# Autodesk Inventor assembly: enix_assembly_v2
(part 2 of 2)
- Mate:543: baseplate:1 ↔ AS 1427 H - Metric M2 x 8:49
- Mate:544: baseplate:1 ↔ AS 1427 H - Metric M2 x 8:49
- Mate:545: baseplate:1 ↔ AS 1427 H - Metric M2 x 8:50
- Mate:546: battery_distancer:2 ↔ AS 1112 (2) - Metric M2  Type 5:54
- Mate:547: AS 1427 H - Metric M2 x 8:50 ↔ AS 1112 (2) - Metric M2  Type 5:54
- Mate:548: battery_distancer:1 ↔ AS 1112 (2) - Metric M2  Type 5:53
- Mate:549: AS 1427 H - Metric M2 x 8:49 ↔ AS 1112 (2) - Metric M2  Type 5:53
- Mate:550: battery_distancer:1 ↔ AS 1112 (2) - Metric M2  Type 5:52
- Mate:551: AS 1427 H - Metric M2 x 8:48 ↔ AS 1112 (2) - Metric M2  Type 5:52
- Mate:552: battery_distancer:2 ↔ AS 1112 (2) - Metric M2  Type 5:51
- Mate:553: AS 1427 H - Metric M2 x 8:47 ↔ AS 1112 (2) - Metric M2  Type 5:51
- Mate:554: battery_distancer:2 ↔ battery_vant_4500_4s:1
- Mate:555 (1 mm): battery_distancer:2 ↔ battery_vant_4500_4s:1
- Mate:556: transformer:1 ↔ AS 1427 H - Metric M2 x 8:51
- Mate:557: transformer:1 ↔ AS 1427 H - Metric M2 x 8:52
- Mate:558: transformer:1 ↔ AS 1427 H - Metric M2 x 8:52
- Mate:559: transformer:1 ↔ AS 1427 H - Metric M2 x 8:51
- Mate:560: transformer:2 ↔ AS 1427 H - Metric M2 x 8:54
- Mate:561: transformer:2 ↔ AS 1427 H - Metric M2 x 8:53
- Mate:562: transformer:2 ↔ AS 1427 H - Metric M2 x 8:53
- Mate:563: transformer:2 ↔ AS 1427 H - Metric M2 x 8:54
- Mate:564: arm_back_rect:2 ↔ motor_mount_lock:4
- Mate:565: arm_front_rect:2 ↔ motor_mount_lock:1
- Mate:566: arm_front_rect:1 ↔ motor_mount_lock:2
- Mate:567: arm_back_rect:1 ↔ motor_mount_lock:3
- Mate:568: arm_back_rect:2 ↔ arm_socket_l:1
- Mate:569: arm_back_rect:2 ↔ arm_socket_l:1
- Mate:570 (0.05 mm): arm_back_rect:2 ↔ arm_socket_l:1
- Mate:571: arm_front_rect:2 ↔ arm_socket_l:2
- Mate:572: arm_front_rect:2 ↔ arm_socket_l:2
- Mate:573 (0.05 mm): arm_front_rect:2 ↔ arm_socket_l:2
- Mate:574: baseplate:1 ↔ arm_socket_l:1
- Mate:575: baseplate:1 ↔ arm_socket_l:1
- Angle:9 (0 deg): baseplate:1 ↔ arm_back_rect:2
- Mate:576: baseplate:1 ↔ arm_socket_l:2
- Mate:577: baseplate:1 ↔ arm_socket_l:2
- Angle:10 (0 deg): baseplate:1 ↔ arm_front_rect:2
- Mate:578: arm_back_rect:1 ↔ arm_socket_r:1
- Mate:579 (0.05 mm): arm_back_rect:1 ↔ arm_socket_r:1
- Mate:580: arm_back_rect:1 ↔ arm_socket_r:1
- Mate:581: arm_front_rect:1 ↔ arm_socket_r:2
- Mate:582 (0.05 mm): arm_front_rect:1 ↔ arm_socket_r:2
- Mate:583: arm_front_rect:1 ↔ arm_socket_r:2
- Mate:584: baseplate:1 ↔ arm_socket_r:2
- Mate:585: baseplate:1 ↔ arm_socket_r:2
- Angle:11 (0 deg): baseplate:1 ↔ arm_front_rect:1
- Mate:586: baseplate:1 ↔ arm_socket_r:1
- Mate:587: baseplate:1 ↔ arm_socket_r:1
- Angle:12 (0 deg): baseplate:1 ↔ arm_back_rect:1
- Mate:588: motor_mount:2 ↔ AS 1112 (2) - Metric M2  Type 5:55
- Mate:589: motor_mount:2 ↔ AS 1112 (2) - Metric M2  Type 5:55
- Mate:590: motor_mount:2 ↔ AS 1112 (2) - Metric M2  Type 5:56
- Mate:591: motor_mount:2 ↔ AS 1112 (2) - Metric M2  Type 5:56
- Mate:592: motor_mount:1 ↔ AS 1112 (2) - Metric M2  Type 5:61
- Mate:593: motor_mount:1 ↔ AS 1112 (2) - Metric M2  Type 5:61
- Mate:594: motor_mount:1 ↔ AS 1112 (2) - Metric M2  Type 5:62
- Mate:595: motor_mount:1 ↔ AS 1112 (2) - Metric M2  Type 5:62
- Mate:596: motor_mount:4 ↔ AS 1112 (2) - Metric M2  Type 5:60
- Mate:597: motor_mount:4 ↔ AS 1112 (2) - Metric M2  Type 5:60
- Mate:598: motor_mount:4 ↔ AS 1112 (2) - Metric M2  Type 5:59
- Mate:599: motor_mount:4 ↔ AS 1112 (2) - Metric M2  Type 5:59
- Mate:600: motor_mount:3 ↔ AS 1112 (2) - Metric M2  Type 5:57
- Mate:601: motor_mount:3 ↔ AS 1112 (2) - Metric M2  Type 5:57
- Mate:602: motor_mount:3 ↔ AS 1112 (2) - Metric M2  Type 5:58
- Mate:603: motor_mount:3 ↔ AS 1112 (2) - Metric M2  Type 5:58
- Mate:604: motor_mount_lock:3 ↔ AS 1427 H - Metric M2 x 12:1
- Mate:605: motor_mount_lock:3 ↔ AS 1427 H - Metric M2 x 12:1
- Mate:606: motor_mount_lock:3 ↔ AS 1427 H - Metric M2 x 12:2
- Mate:607: motor_mount_lock:3 ↔ AS 1427 H - Metric M2 x 12:2
- Mate:608: motor_mount_lock:4 ↔ AS 1427 H - Metric M2 x 12:5
- Mate:609: motor_mount_lock:4 ↔ AS 1427 H - Metric M2 x 12:5
- Mate:610: motor_mount_lock:4 ↔ AS 1427 H - Metric M2 x 12:6
- Mate:611: motor_mount_lock:4 ↔ AS 1427 H - Metric M2 x 12:6
- Mate:612: motor_mount_lock:1 ↔ AS 1427 H - Metric M2 x 12:8
- Mate:613: motor_mount_lock:1 ↔ AS 1427 H - Metric M2 x 12:8
- Mate:614: motor_mount_lock:1 ↔ AS 1427 H - Metric M2 x 12:7
- Mate:615: motor_mount_lock:1 ↔ AS 1427 H - Metric M2 x 12:7
- Mate:616: motor_mount_lock:2 ↔ AS 1427 H - Metric M2 x 12:3
- Mate:617: motor_mount_lock:2 ↔ AS 1427 H - Metric M2 x 12:3
- Mate:618: motor_mount_lock:2 ↔ AS 1427 H - Metric M2 x 12:4
- Mate:619: motor_mount_lock:2 ↔ AS 1427 H - Metric M2 x 12:4
- Mate:620: motor_mount_lock:2 ↔ AS 1427 H - Metric M3 x 10:1
- Mate:621: motor_mount_lock:2 ↔ AS 1427 H - Metric M3 x 10:1
- Mate:622: arm_front_rect:1 ↔ ANSI B18.2.4.2M M3x0,5:1
- Mate:623: AS 1427 H - Metric M3 x 10:1 ↔ ANSI B18.2.4.2M M3x0,5:1
- Mate:624: motor_mount_lock:3 ↔ AS 1427 H - Metric M3 x 10:2
- Mate:625: motor_mount_lock:3 ↔ AS 1427 H - Metric M3 x 10:2
- Mate:626: motor_mount_lock:4 ↔ AS 1427 H - Metric M3 x 10:3
- Mate:627: motor_mount_lock:4 ↔ AS 1427 H - Metric M3 x 10:3
- Mate:628: motor_mount_lock:1 ↔ AS 1427 H - Metric M3 x 10:4
- Mate:629: motor_mount_lock:1 ↔ AS 1427 H - Metric M3 x 10:4
- Mate:630: arm_back_rect:1 ↔ ANSI B18.2.4.2M M3x0,5:2
- Mate:631: AS 1427 H - Metric M3 x 10:2 ↔ ANSI B18.2.4.2M M3x0,5:2
- Mate:632: arm_back_rect:2 ↔ ANSI B18.2.4.2M M3x0,5:3
- Mate:633: AS 1427 H - Metric M3 x 10:3 ↔ ANSI B18.2.4.2M M3x0,5:3
- Mate:634: arm_front_rect:2 ↔ ANSI B18.2.4.2M M3x0,5:4
- Mate:635: AS 1427 H - Metric M3 x 10:4 ↔ ANSI B18.2.4.2M M3x0,5:4
- Mate:636: motor_mount:3 ↔ Emax Rs2205 v1:4
- Mate:637: motor_mount:3 ↔ Emax Rs2205 v1:4
- Mate:638: motor_mount:3 ↔ Emax Rs2205 v1:4
- Mate:639: motor_mount:3 ↔ AS 1427 H - Metric M3 x 5:21
- Mate:640: motor_mount:3 ↔ AS 1427 H - Metric M3 x 5:21
- Mate:641: motor_mount:3 ↔ AS 1427 H - Metric M3 x 5:24
- Mate:642: motor_mount:3 ↔ AS 1427 H - Metric M3 x 5:24
- Mate:643: motor_mount:3 ↔ AS 1427 H - Metric M3 x 5:23
- Mate:644: motor_mount:3 ↔ AS 1427 H - Metric M3 x 5:23
- Mate:645: motor_mount:3 ↔ AS 1427 H - Metric M3 x 5:22
- Mate:646: motor_mount:3 ↔ AS 1427 H - Metric M3 x 5:22
- Mate:647: motor_mount:4 ↔ AS 1427 H - Metric M3 x 5:33
- Mate:648: motor_mount:4 ↔ AS 1427 H - Metric M3 x 5:33
- Mate:649: motor_mount:4 ↔ AS 1427 H - Metric M3 x 5:34
- Mate:650: motor_mount:4 ↔ AS 1427 H - Metric M3 x 5:34
- Mate:651: motor_mount:4 ↔ AS 1427 H - Metric M3 x 5:35
- Mate:652: motor_mount:4 ↔ AS 1427 H - Metric M3 x 5:35
- Mate:653: motor_mount:4 ↔ AS 1427 H - Metric M3 x 5:36
- Mate:654: motor_mount:4 ↔ AS 1427 H - Metric M3 x 5:36
- Mate:655: motor_mount:4 ↔ Emax Rs2205 v1:3
- Mate:656: Emax Rs2205 v1:3 ↔ AS 1427 H - Metric M3 x 5:33
- Mate:657: Emax Rs2205 v1:3 ↔ AS 1427 H - Metric M3 x 5:34
- Mate:658: motor_mount:1 ↔ AS 1427 H - Metric M3 x 5:27
- Mate:659: motor_mount:1 ↔ AS 1427 H - Metric M3 x 5:26
- Mate:660: motor_mount:1 ↔ AS 1427 H - Metric M3 x 5:25
- Mate:661: motor_mount:1 ↔ AS 1427 H - Metric M3 x 5:28
- Mate:662: motor_mount:1 ↔ AS 1427 H - Metric M3 x 5:27
- Mate:663: motor_mount:1 ↔ AS 1427 H - Metric M3 x 5:26
- Mate:664: motor_mount:1 ↔ AS 1427 H - Metric M3 x 5:25
- Mate:665: motor_mount:1 ↔ AS 1427 H - Metric M3 x 5:28
- Mate:666: motor_mount:1 ↔ Emax Rs2205 v1:2
- Mate:667: Emax Rs2205 v1:2 ↔ AS 1427 H - Metric M3 x 5:26
- Mate:668: Emax Rs2205 v1:2 ↔ AS 1427 H - Metric M3 x 5:27
- Mate:669: motor_mount:2 ↔ AS 1427 H - Metric M3 x 5:31
- Mate:670: motor_mount:2 ↔ AS 1427 H - Metric M3 x 5:32
- Mate:671: motor_mount:2 ↔ AS 1427 H - Metric M3 x 5:29
- Mate:672: motor_mount:2 ↔ AS 1427 H - Metric M3 x 5:30
- Mate:673: motor_mount:2 ↔ AS 1427 H - Metric M3 x 5:30
- Mate:674: motor_mount:2 ↔ AS 1427 H - Metric M3 x 5:31
- Mate:675: motor_mount:2 ↔ AS 1427 H - Metric M3 x 5:29
- Mate:676: motor_mount:2 ↔ AS 1427 H - Metric M3 x 5:32
- Mate:677: motor_mount:2 ↔ Emax Rs2205 v1:1
- Mate:678: Emax Rs2205 v1:1 ↔ AS 1427 H - Metric M3 x 5:32
- Mate:679: Emax Rs2205 v1:1 ↔ AS 1427 H - Metric M3 x 5:29
- Mate:680: top_plate:1 ↔ AS 1427 H - Metric M2 x 8:55
- Mate:681: top_plate:1 ↔ AS 1427 H - Metric M2 x 8:57
- Mate:682: top_plate:1 ↔ AS 1427 H - Metric M2 x 8:56
- Mate:683: top_plate:1 ↔ AS 1427 H - Metric M2 x 8:59
- Mate:684: arm_socket_l:1 ↔ AS 1427 H - Metric M2 x 8:58
- Mate:685: arm_socket_l:1 ↔ AS 1427 H - Metric M2 x 8:60
- Mate:686: arm_socket_l:2 ↔ AS 1427 H - Metric M2 x 8:62
- Mate:687: arm_socket_l:2 ↔ AS 1427 H - Metric M2 x 8:61
- Mate:688: arm_socket_l:2 ↔ AS 1427 H - Metric M2 x 8:61
- Mate:689: arm_socket_l:2 ↔ AS 1427 H - Metric M2 x 8:62
- Mate:690: top_plate:1 ↔ AS 1427 H - Metric M2 x 8:55
- Mate:691: top_plate:1 ↔ AS 1427 H - Metric M2 x 8:57
- Mate:692: top_plate:1 ↔ AS 1427 H - Metric M2 x 8:69
- Mate:693: top_plate:1 ↔ AS 1427 H - Metric M2 x 8:70
- Mate:694: arm_socket_r:2 ↔ AS 1427 H - Metric M2 x 8:68
- Mate:695: arm_socket_r:2 ↔ AS 1427 H - Metric M2 x 8:67
- Mate:696: top_plate:1 ↔ AS 1427 H - Metric M2 x 8:66
- Mate:697: top_plate:1 ↔ AS 1427 H - Metric M2 x 8:65
- Mate:698: arm_socket_r:1 ↔ AS 1427 H - Metric M2 x 8:64
- Mate:699: arm_socket_r:1 ↔ AS 1427 H - Metric M2 x 8:63
- Mate:700: arm_socket_r:1 ↔ AS 1427 H - Metric M2 x 8:64
- Mate:701: top_plate:1 ↔ AS 1427 H - Metric M2 x 8:66
- Mate:702: top_plate:1 ↔ AS 1427 H - Metric M2 x 8:65
- Mate:703: arm_socket_r:1 ↔ AS 1427 H - Metric M2 x 8:63
- Mate:704: top_plate:1 ↔ AS 1427 H - Metric M2 x 8:59
- Mate:705: top_plate:1 ↔ AS 1427 H - Metric M2 x 8:56
- Mate:706: arm_socket_l:1 ↔ AS 1427 H - Metric M2 x 8:58
- Mate:707: arm_socket_l:1 ↔ AS 1427 H - Metric M2 x 8:60
- Mate:708: top_plate:1 ↔ AS 1427 H - Metric M2 x 8:70
- Mate:709: top_plate:1 ↔ AS 1427 H - Metric M2 x 8:69
- Mate:710: arm_socket_r:2 ↔ AS 1427 H - Metric M2 x 8:68
- Mate:711: arm_socket_r:2 ↔ AS 1427 H - Metric M2 x 8:67
- Mate:712: baseplate:1 ↔ AS 1112 (2) - Metric M2  Type 5:66
- Mate:713: baseplate:1 ↔ AS 1112 (2) - Metric M2  Type 5:65
- Mate:714: AS 1427 H - Metric M2 x 8:63 ↔ AS 1112 (2) - Metric M2  Type 5:65
- Mate:715: AS 1427 H - Metric M2 x 8:64 ↔ AS 1112 (2) - Metric M2  Type 5:66
- Mate:716: arm_socket_r:1 ↔ AS 1112 (2) - Metric M2  Type 5:64
- Mate:717: AS 1427 H - Metric M2 x 8:66 ↔ AS 1112 (2) - Metric M2  Type 5:64
- Mate:718: arm_socket_r:1 ↔ AS 1112 (2) - Metric M2  Type 5:63
- Mate:719: AS 1427 H - Metric M2 x 8:65 ↔ AS 1112 (2) - Metric M2  Type 5:63
- Mate:720: arm_socket_r:2 ↔ AS 1112 (2) - Metric M2  Type 5:67
- Mate:721: AS 1427 H - Metric M2 x 8:69 ↔ AS 1112 (2) - Metric M2  Type 5:67
- Mate:722: arm_socket_r:2 ↔ AS 1112 (2) - Metric M2  Type 5:70
- Mate:723: AS 1427 H - Metric M2 x 8:70 ↔ AS 1112 (2) - Metric M2  Type 5:70
- Mate:724: baseplate:1 ↔ AS 1112 (2) - Metric M2  Type 5:69
- Mate:725: baseplate:1 ↔ AS 1112 (2) - Metric M2  Type 5:68
- Mate:726: AS 1427 H - Metric M2 x 8:67 ↔ AS 1112 (2) - Metric M2  Type 5:68
- Mate:727: AS 1427 H - Metric M2 x 8:68 ↔ AS 1112 (2) - Metric M2  Type 5:69
- Mate:728: arm_socket_l:1 ↔ AS 1112 (2) - Metric M2  Type 5:77
- Mate:729: AS 1427 H - Metric M2 x 8:56 ↔ AS 1112 (2) - Metric M2  Type 5:77
- Mate:730: arm_socket_l:1 ↔ AS 1112 (2) - Metric M2  Type 5:75
- Mate:731: AS 1427 H - Metric M2 x 8:59 ↔ AS 1112 (2) - Metric M2  Type 5:75
- Mate:732: baseplate:1 ↔ AS 1112 (2) - Metric M2  Type 5:78
- Mate:733: baseplate:1 ↔ AS 1112 (2) - Metric M2  Type 5:76
- Mate:734: AS 1427 H - Metric M2 x 8:60 ↔ AS 1112 (2) - Metric M2  Type 5:76
- Mate:735: AS 1427 H - Metric M2 x 8:58 ↔ AS 1112 (2) - Metric M2  Type 5:78
- Mate:736: arm_socket_l:2 ↔ AS 1112 (2) - Metric M2  Type 5:71
- Mate:737: AS 1427 H - Metric M2 x 8:55 ↔ AS 1112 (2) - Metric M2  Type 5:71
- Mate:738: baseplate:1 ↔ AS 1112 (2) - Metric M2  Type 5:72
- Mate:739: AS 1427 H - Metric M2 x 8:62 ↔ AS 1112 (2) - Metric M2  Type 5:72
- Mate:740: baseplate:1 ↔ AS 1112 (2) - Metric M2  Type 5:74
- Mate:741: AS 1427 H - Metric M2 x 8:61 ↔ AS 1112 (2) - Metric M2  Type 5:74
- Mate:742: arm_socket_l:2 ↔ AS 1112 (2) - Metric M2  Type 5:73
- Mate:743: AS 1427 H - Metric M2 x 8:57 ↔ AS 1112 (2) - Metric M2  Type 5:73
- Mate:744: top_plate:1 ↔ AS 1427 H - Metric M3 x 30:1
- Mate:745: top_plate:1 ↔ AS 1427 H - Metric M3 x 30:1
- Mate:746: top_plate:1 ↔ AS 1427 H - Metric M3 x 30:2
- Mate:747: top_plate:1 ↔ AS 1427 H - Metric M3 x 30:4
- Mate:748: top_plate:1 ↔ AS 1427 H - Metric M3 x 30:3
- Mate:749: top_plate:1 ↔ AS 1427 H - Metric M3 x 30:3
- Mate:750: top_plate:1 ↔ AS 1427 H - Metric M3 x 30:4
- Mate:751: top_plate:1 ↔ AS 1427 H - Metric M3 x 30:2
- Mate:752: baseplate:1 ↔ ANSI B18.2.4.2M M3x0,5:8
- Mate:753: baseplate:1 ↔ ANSI B18.2.4.2M M3x0,5:6
- Mate:754: AS 1427 H - Metric M3 x 30:2 ↔ ANSI B18.2.4.2M M3x0,5:6
- Mate:755: AS 1427 H - Metric M3 x 30:1 ↔ ANSI B18.2.4.2M M3x0,5:8
- Mate:756: baseplate:1 ↔ ANSI B18.2.4.2M M3x0,5:5
- Mate:757: baseplate:1 ↔ ANSI B18.2.4.2M M3x0,5:5
- Mate:758: baseplate:1 ↔ ANSI B18.2.4.2M M3x0,5:7
- Mate:759: AS 1427 H - Metric M3 x 30:4 ↔ ANSI B18.2.4.2M M3x0,5:7
- Mate:760: top_plate:1 ↔ klatka_na_rpi:1
- Mate:761: top_plate:1 ↔ klatka_na_rpi:1
- Mate:762: top_plate:1 ↔ klatka_na_rpi:1
- Mate:763: top_plate:1 ↔ klatka_na_rpi:1
- Mate:764: klatka_na_rpi:1 ↔ AS 1427 H - Metric M2 x 8:73
- Mate:765: klatka_na_rpi:1 ↔ AS 1427 H - Metric M2 x 8:72
- Mate:766: klatka_na_rpi:1 ↔ AS 1427 H - Metric M2 x 8:71
- Mate:767: klatka_na_rpi:1 ↔ AS 1427 H - Metric M2 x 8:71
- Mate:768: klatka_na_rpi:1 ↔ AS 1427 H - Metric M2 x 8:72
- Mate:769: klatka_na_rpi:1 ↔ AS 1427 H - Metric M2 x 8:73
- Mate:770: klatka_na_rpi:1 ↔ AS 1427 H - Metric M2 x 8:76
- Mate:771: klatka_na_rpi:1 ↔ AS 1427 H - Metric M2 x 8:75
- Mate:772: klatka_na_rpi:1 ↔ AS 1427 H - Metric M2 x 8:74
- Mate:773: klatka_na_rpi:1 ↔ AS 1427 H - Metric M2 x 8:74
- Mate:774: klatka_na_rpi:1 ↔ AS 1427 H - Metric M2 x 8:75
- Mate:775: klatka_na_rpi:1 ↔ AS 1427 H - Metric M2 x 8:76
- Mate:776: top_plate:1 ↔ AS 1112 (2) - Metric M2  Type 5:80
- Mate:777: AS 1427 H - Metric M2 x 8:72 ↔ AS 1112 (2) - Metric M2  Type 5:80
- Mate:778: top_plate:1 ↔ AS 1112 (2) - Metric M2  Type 5:81
- Mate:779: AS 1427 H - Metric M2 x 8:71 ↔ AS 1112 (2) - Metric M2  Type 5:81
- Mate:780: top_plate:1 ↔ AS 1112 (2) - Metric M2  Type 5:79
- Mate:781: AS 1427 H - Metric M2 x 8:73 ↔ AS 1112 (2) - Metric M2  Type 5:79
- Mate:782: top_plate:1 ↔ AS 1112 (2) - Metric M2  Type 5:84
- Mate:783: AS 1427 H - Metric M2 x 8:76 ↔ AS 1112 (2) - Metric M2  Type 5:84
- Mate:784: top_plate:1 ↔ AS 1112 (2) - Metric M2  Type 5:83
- Mate:785: AS 1427 H - Metric M2 x 8:75 ↔ AS 1112 (2) - Metric M2  Type 5:83
- Mate:786: top_plate:1 ↔ AS 1112 (2) - Metric M2  Type 5:82
- Mate:787: top_plate:1 ↔ AS 1112 (2) - Metric M2  Type 5:82
## Named parameters: sa_0 = -13.8611, sa_1 = 0, sa_2 = 999.904, sa_3 = -5.52663, sa_4 = 0, sa_5 = 999.985, sa_6 = 0, sa_7 = -500, sa_8 = -0
note: some values were not read from the file. Shown as the stored number, unit unknown: "sa_0", "sa_1", "sa_2", "sa_3", "sa_4", "sa_5", "sa_6", "sa_7", "sa_8".
